# Autodesk Inventor assembly: NF-A9x14 PWM
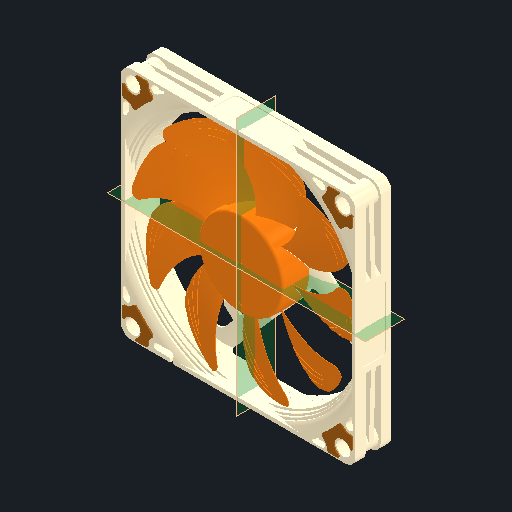
[picture p0: Inventor's stored thumbnail of the model, 512x512]
Saved by Autodesk Inventor 2026.1 (Build 301233020, 233B)
## iProperties
Created: 2022-09-10
Part Number: NF-A9x14 PWM
Description: STEP AP214
Document SubType Name: Assembly
Designer: atrus
Sending System: SolidWorks 2022
Preprocessor: SwSTEP 2.0
Title: NF-A9x14 PWM.STEP
Revision Number: ANY
## Documents named in this file (11)
- C:\Users\atrus\Dropbox\elec\Mechanical\LEDBrick\NF-A9x14 PWM\NF-A9x14 PWM\NF-A9x14 PWM.iam
- C:\Users\atrus\Dropbox\elec\Mechanical\LEDBrick\NF-A9x14 PWM\NF-A9x14 PWM\Case A9x14_Predeterminado.ipt
- C:\Users\atrus\Dropbox\elec\Mechanical\LEDBrick\NF-A9x14 PWM\NF-A9x14 PWM\Silent block A9x14_Predeterminado.ipt
- C:\Users\atrus\Dropbox\elec\Mechanical\LEDBrick\NF-A9x14 PWM\NF-A9x14 PWM\Magnet A9x14_Predeterminado.ipt
- C:\Users\atrus\Dropbox\elec\Mechanical\LEDBrick\NF-A9x14 PWM\NF-A9x14 PWM\Back plate A9x14_Predeterminado.ipt
- C:\Users\atrus\Dropbox\elec\Mechanical\LEDBrick\NF-A9x14 PWM\NF-A9x14 PWM\Impeller A9x14_Predeterminado.ipt
- C:\Users\atrus\Dropbox\elec\Mechanical\LEDBrick\NF-A9x14 PWM\NF-A9x14 PWM\Magnetic screen A9x14_Predeterminado.ipt
- C:\Users\atrus\Dropbox\elec\Mechanical\LEDBrick\NF-A9x14 PWM\NF-A9x14 PWM\Rotor A9x14_Predeterminado.ipt
- C:\Users\atrus\Dropbox\elec\Mechanical\LEDBrick\NF-A9x14 PWM\NF-A9x14 PWM\Shaft A9x14_Predeterminado.ipt
- C:\Users\atrus\Dropbox\elec\Mechanical\LEDBrick\NF-A9x14 PWM\NF-A9x14 PWM\Oil Bearing A9x14_Predeterminado.iam
- C:\Users\atrus\Dropbox\elec\Mechanical\LEDBrick\NF-A9x14 PWM\NF-A9x14 PWM\Brushless motor A9x14_Predeterminado.iam
## Components (17 placed, 17 different names)
1. Case A9x14_Predeterminado_1 — Flush:1, Flush:2
2. Silent block A9x14_Predeterminado_2
3. Silent block A9x14_Predeterminado_3
4. Silent block A9x14_Predeterminado_4
5. Silent block A9x14_Predeterminado_5
6. Silent block A9x14_Predeterminado_6
7. Silent block A9x14_Predeterminado_7
8. Silent block A9x14_Predeterminado_8
9. Silent block A9x14_Predeterminado_9
10. Magnet A9x14_Predeterminado_10
11. Back plate A9x14_Predeterminado_11
12. Impeller A9x14_Predeterminado_12
13. Magnetic screen A9x14_Predeterminado_13
14. Rotor A9x14_Predeterminado_14
15. Shaft A9x14_Predeterminado_15
16. Oil Bearing A9x14_Predeterminado_16 [sub-assembly]
17. Brushless motor A9x14_Predeterminado_17 [sub-assembly]
## Relationships (2: Flush 2)
- Flush:1 (-46 mm): Case A9x14_Predeterminado_1
- Flush:2 (-46 mm): Case A9x14_Predeterminado_1
